# Autodesk Inventor assembly: Assembly
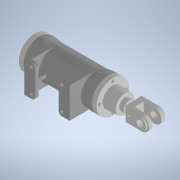
[picture p0: Inventor's stored thumbnail of the model, 180x180]
Saved by Autodesk Inventor 2021 (Build 250183000, 183)
## iProperties
Created: 2022-06-06
Part Number: Assembly
Document SubType Name: Assembly
Designer: Bhargav Malasani
Author: Bhargav Malasani
## Documents named in this file (9)
- E:\final\Assembly.iam
- E:\final\Part1.ipt
- E:\final\Part2.ipt
- E:\final\Part3.ipt
- E:\final\Part4.ipt
- E:\final\Part5.ipt
- E:\final\Part6.ipt
- E:\final\Part7.ipt
- E:\final\Part8.ipt
## Components (8 placed, 8 different names)
1. Part1:1 — Mate:1, Mate:2, Mate:3, Insert:1, Mate:11, Mate:13, Mate:14
2. Part2:1 — Mate:1, Mate:2, Mate:3
3. Part3:1 — Insert:2, Mate:4
4. Part4:1 — Mate:9, Mate:10, Mate:12
5. Part5:1 — Insert:3
6. Part6:1 — Mate:8
7. Part7:1 — Insert:1, Insert:2, Mate:4, Insert:3, Mate:8
8. Part8:1 — Mate:9, Mate:10, Mate:11, Mate:12, Mate:13, Mate:14
## Relationships (14: Mate 11, Insert 3)
- Mate:1: Part1:1 ↔ Part2:1
- Mate:2: Part1:1 ↔ Part2:1
- Mate:3: Part1:1 ↔ Part2:1
- Insert:1: Part1:1 ↔ Part7:1
- Insert:2 (-1 mm): Part3:1 ↔ Part7:1
- Mate:4 (2 mm): Part3:1 ↔ Part7:1
- Insert:3 (-27.4 mm): Part5:1 ↔ Part7:1
- Mate:8 (12 mm): Part6:1 ↔ Part7:1
- Mate:9: Part4:1 ↔ Part8:1
- Mate:10: Part4:1 ↔ Part8:1
- Mate:11: Part1:1 ↔ Part8:1
- Mate:12: Part4:1 ↔ Part8:1
- Mate:13: Part1:1 ↔ Part8:1
- Mate:14: Part1:1 ↔ Part8:1
